# Autodesk Inventor assembly: Leg_joint_yaw_shim_basis
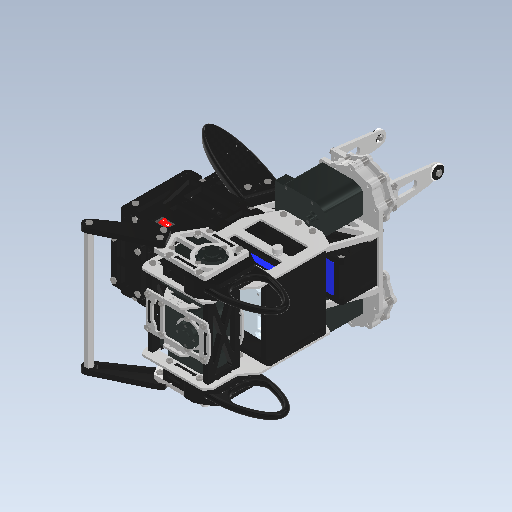
[picture p0: Inventor's stored thumbnail of the model, 512x512]
Saved by Autodesk Inventor 2020 (Build 240168000, 168)
## iProperties
Created: 2021-11-14
Part Number: Leg_joint_yaw_shim_basis
Document SubType Name: Assembly
Designer: Masato Kubotera
Author: Masato Kubotera
## Documents named in this file (3)
- C:\Users\Masato\Documents\Inventor\CIT Brains_Inventor\OpenPlatform_ver3_0\Shim\Leg_joint_yaw_shim_basis.iam
- C:\Users\Masato\Documents\Inventor\CIT Brains_Inventor\OpenPlatform_ver3_0\LowerBody\Leg_joit\Leg_joint_roll_yaw.iam
- C:\Users\Masato\Documents\Inventor\CIT Brains_Inventor\OpenPlatform_ver3_0\UpperBody\Trunk\Trunk.iam
## Components (2 placed, 2 different names)
1. Leg_joint_roll_yaw:1 [sub-assembly] — 挿入:1, 角度:1
2. Trunk:1 [sub-assembly] — 挿入:1, 角度:1
## Relationships (2: Insert 1, Angle 1)
- 挿入:1 [Insert]: Leg_joint_roll_yaw:1 ↔ Trunk:1
- 角度:1 [Angle] (0 deg): Leg_joint_roll_yaw:1 ↔ Trunk:1
